# Autodesk Inventor assembly: BL Motor + Encoder + Gearbox
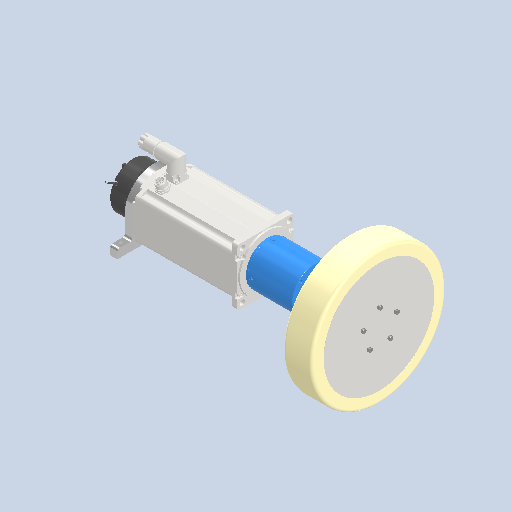
[picture p0: Inventor's stored thumbnail of the model, 512x512]
Saved by Autodesk Inventor 2022.1 (Build 261234000, 234)
## iProperties
Created: 2021-09-22
Part Number: BL Motor + Encoder + Gearbox
Document SubType Name: Assembly
Designer: seb_0
Author: seb_0
## Documents named in this file (9)
- C:\Users\seb_0\Desktop\PDM\ProyectoRobotPallet\Motor\BL Motor + Encoder + Gearbox + Rueda.iam
- C:\Users\seb_0\Desktop\PDM\ProyectoRobotPallet\Motor\Encoder - E 600R\e600-8871002100.ipt
- C:\Users\seb_0\Desktop\PDM\ProyectoRobotPallet\Motor\Rueda\Rueda.iam
- C:\Users\seb_0\Desktop\PDM\ProyectoRobotPallet\Motor\Rueda\Sprocket_Rueda.ipt
- C:\Users\seb_0\Desktop\PDM\ProyectoRobotPallet\Motor\BL Motor - BG 95x80 dCore\bg-95x80-885950205312.ipt
- C:\Users\seb_0\Desktop\PDM\ProyectoRobotPallet\Motor\Gearbox - PLG 75 HT 10.1\plg-75-8887505053.ipt
- C:\Users\seb_0\Desktop\PDM\ProyectoRobotPallet\Soportes\Soporte_Motor_Encoder.ipt
- C:\Users\seb_0\Desktop\PDM\ProyectoRobotPallet\ContentCenter\es-ES\ISO 4762(2)\ISO 4762 - M4 x 35ISO.ipt
- C:\Users\seb_0\Desktop\PDM\ProyectoRobotPallet\ContentCenter\es-ES\ISO 4032(2)\ISO 4032 - M4 - ISO.ipt
## Components (16 placed, 8 different names)
1. e600-8871002100:1 — Coincidencia:16, Coincidencia:17, Coincidencia:18, Coincidencia:26
2. Rueda:1 [sub-assembly] — Coincidencia:11, Coincidencia:27, Coincidencia:28, Coincidencia:29, Coincidencia:30, Coincidencia:31, Coincidencia:33, Coincidencia:34, Coincidencia:35, Coincidencia:41, Coincidencia:42, Coincidencia:43, Coincidencia:45, Coincidencia:46, Coincidencia:47, Coincidencia:49, Coincidencia:50, Coincidencia:51
3. Sprocket_Rueda:1 — Coincidencia:11, Coincidencia:22, Coincidencia:23, Coincidencia:24, Coincidencia:27, Coincidencia:28, Coincidencia:32, Coincidencia:36, Coincidencia:44, Coincidencia:48, Coincidencia:52
4. bg-95x80-885950205312:1 — Coincidencia:14, Coincidencia:15, Coincidencia:16, Coincidencia:17, Coincidencia:18, Coincidencia:19, Coincidencia:20, Coincidencia:21, Coincidencia:25, Nivelación:1
5. plg-75-8887505053:1 — Coincidencia:19, Coincidencia:20, Coincidencia:21, Coincidencia:22, Coincidencia:23, Coincidencia:24
6. Soporte_Motor_Encoder:1 — Coincidencia:25, Coincidencia:26, Nivelación:1
7. ISO 4762 M4 x 35:1 — Coincidencia:29, Coincidencia:30
8. ISO 4032 M4:1 — Coincidencia:31, Coincidencia:32
9. ISO 4762 M4 x 35:2 — Coincidencia:33, Coincidencia:34
10. ISO 4032 M4:2 — Coincidencia:35, Coincidencia:36
11. ISO 4762 M4 x 35:3 — Coincidencia:41, Coincidencia:42
12. ISO 4032 M4:3 — Coincidencia:43, Coincidencia:44
13. ISO 4762 M4 x 35:4 — Coincidencia:45, Coincidencia:46
14. ISO 4032 M4:4 — Coincidencia:47, Coincidencia:48
15. ISO 4762 M4 x 35:5 — Coincidencia:49, Coincidencia:50
16. ISO 4032 M4:5 — Coincidencia:51, Coincidencia:52
## Relationships (37: Mate 36, Flush 1)
- Coincidencia:11 [Mate]: Rueda:1 ↔ Sprocket_Rueda:1
- Coincidencia:14 [Mate]: bg-95x80-885950205312:1
- Coincidencia:15 [Mate]: bg-95x80-885950205312:1
- Coincidencia:16 [Mate]: e600-8871002100:1 ↔ bg-95x80-885950205312:1
- Coincidencia:17 [Mate]: e600-8871002100:1 ↔ bg-95x80-885950205312:1
- Coincidencia:18 [Mate]: e600-8871002100:1 ↔ bg-95x80-885950205312:1
- Coincidencia:19 [Mate]: bg-95x80-885950205312:1 ↔ plg-75-8887505053:1
- Coincidencia:20 [Mate]: bg-95x80-885950205312:1 ↔ plg-75-8887505053:1
- Coincidencia:21 [Mate] (-34.858 mm): bg-95x80-885950205312:1 ↔ plg-75-8887505053:1
- Coincidencia:22 [Mate]: Sprocket_Rueda:1 ↔ plg-75-8887505053:1
- Coincidencia:23 [Mate]: Sprocket_Rueda:1 ↔ plg-75-8887505053:1
- Coincidencia:24 [Mate] (5 mm): Sprocket_Rueda:1 ↔ plg-75-8887505053:1
- Coincidencia:25 [Mate]: bg-95x80-885950205312:1 ↔ Soporte_Motor_Encoder:1
- Coincidencia:26 [Mate]: e600-8871002100:1 ↔ Soporte_Motor_Encoder:1
- Nivelación:1 [Flush] (-0.5 mm): bg-95x80-885950205312:1 ↔ Soporte_Motor_Encoder:1
- Coincidencia:27 [Mate]: Rueda:1 ↔ Sprocket_Rueda:1
- Coincidencia:28 [Mate]: Rueda:1 ↔ Sprocket_Rueda:1
- Coincidencia:29 [Mate]: Rueda:1 ↔ ISO 4762 M4 x 35:1
- Coincidencia:30 [Mate]: Rueda:1 ↔ ISO 4762 M4 x 35:1
- Coincidencia:31 [Mate]: Rueda:1 ↔ ISO 4032 M4:1
- Coincidencia:32 [Mate]: Sprocket_Rueda:1 ↔ ISO 4032 M4:1
- Coincidencia:33 [Mate]: Rueda:1 ↔ ISO 4762 M4 x 35:2
- Coincidencia:34 [Mate]: Rueda:1 ↔ ISO 4762 M4 x 35:2
- Coincidencia:35 [Mate]: Rueda:1 ↔ ISO 4032 M4:2
- Coincidencia:36 [Mate]: Sprocket_Rueda:1 ↔ ISO 4032 M4:2
- Coincidencia:41 [Mate]: Rueda:1 ↔ ISO 4762 M4 x 35:3
- Coincidencia:42 [Mate]: Rueda:1 ↔ ISO 4762 M4 x 35:3
- Coincidencia:43 [Mate]: Rueda:1 ↔ ISO 4032 M4:3
- Coincidencia:44 [Mate]: Sprocket_Rueda:1 ↔ ISO 4032 M4:3
- Coincidencia:45 [Mate]: Rueda:1 ↔ ISO 4762 M4 x 35:4
- Coincidencia:46 [Mate]: Rueda:1 ↔ ISO 4762 M4 x 35:4
- Coincidencia:47 [Mate]: Rueda:1 ↔ ISO 4032 M4:4
- Coincidencia:48 [Mate]: Sprocket_Rueda:1 ↔ ISO 4032 M4:4
- Coincidencia:49 [Mate]: Rueda:1 ↔ ISO 4762 M4 x 35:5
- Coincidencia:50 [Mate]: Rueda:1 ↔ ISO 4762 M4 x 35:5
- Coincidencia:51 [Mate]: Rueda:1 ↔ ISO 4032 M4:5
- Coincidencia:52 [Mate]: Sprocket_Rueda:1 ↔ ISO 4032 M4:5
